# Autodesk Inventor assembly: アームアセンブリ
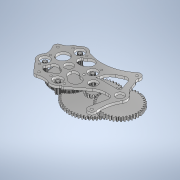
[picture p0: Inventor's stored thumbnail of the model, 180x180]
Saved by Autodesk Inventor 2022.2 (Build 262287030, 287C)
## iProperties
Created: 2022-03-06
Part Number: アームアセンブリ
Document SubType Name: Assembly
Designer: acps
Author: acps
## Documents named in this file (8)
- C:\Users\acps\Documents\srdc\srdc_ksh\アーム\アームアセンブリ.iam
- C:\Users\acps\Documents\srdc\srdc_ksh\アーム\モータマウント.ipt
- C:\Users\acps\Documents\srdc\srdc_ksh\アーム\ギア\ぴにょん歯数8.ipt
- C:\Users\acps\Documents\srdc\srdc_ksh\アーム\ギア\初段焼結歯数80.ipt
- C:\Users\acps\Documents\srdc\srdc_ksh\アーム\ギア\初段多段部分歯数7.ipt
- C:\Users\acps\Documents\srdc\srdc_ksh\アーム\ギア\二段歯数57.ipt
- C:\Users\acps\Documents\srdc\srdc_ksh\アーム\ギア\二段多段部分歯数14.ipt
- C:\Users\acps\Documents\srdc\srdc_ksh\アーム\ギア\最終段歯数43.ipt
## Components (10 placed, 7 different names)
1. モータマウント:1 — Mate:1, Mate:2, Mate:3, Mate:4, Mate:5, Mate:7, Mate:8, Mate:9
2. ぴにょん歯数8:1 — Mate:1
3. ぴにょん歯数8:2 — Mate:2
4. ぴにょん歯数8:3 — Mate:3
5. ぴにょん歯数8:4 — Mate:4
6. 初段焼結歯数80:1 — Mate:5, Mate:6
7. 初段多段部分歯数7:1 — Mate:6
8. 二段歯数57:1 — Mate:7
9. 二段多段部分歯数14:1 — Mate:8
10. 最終段歯数43:1 — Mate:9
## Relationships (9: Mate 9)
- Mate:1: モータマウント:1 ↔ ぴにょん歯数8:1
- Mate:2: モータマウント:1 ↔ ぴにょん歯数8:2
- Mate:3: モータマウント:1 ↔ ぴにょん歯数8:3
- Mate:4: モータマウント:1 ↔ ぴにょん歯数8:4
- Mate:5: モータマウント:1 ↔ 初段焼結歯数80:1
- Mate:6: 初段焼結歯数80:1 ↔ 初段多段部分歯数7:1
- Mate:7: モータマウント:1 ↔ 二段歯数57:1
- Mate:8: モータマウント:1 ↔ 二段多段部分歯数14:1
- Mate:9: モータマウント:1 ↔ 最終段歯数43:1
